# Autodesk Inventor assembly: arm_put_together
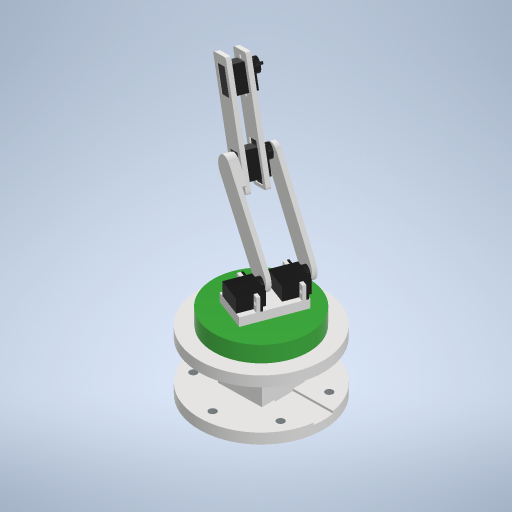
[picture p0: Inventor's stored thumbnail of the model, 512x512]
Saved by Autodesk Inventor 2023 (Build 270158000, 158)
## iProperties
Created: 2023-02-26
Part Number: arm_put_together
Document SubType Name: Assembly
Designer: kamil
Author: kamil
## Documents named in this file (12)
- C:\Users\kamil\Desktop\robotic arm\Inventor_parts\arm_put_together.iam
- C:\Users\kamil\Desktop\robotic arm\Inventor_parts\Base_bottom.ipt
- C:\Users\kamil\Desktop\robotic arm\Inventor_parts\Stepper_model.ipt
- C:\Users\kamil\Desktop\robotic arm\Inventor_parts\Base_top.ipt
- C:\Users\kamil\Desktop\robotic arm\Inventor_parts\Bearing_ball.ipt
- C:\Users\kamil\Desktop\robotic arm\Inventor_parts\Base_arm_mount.ipt
- C:\Users\kamil\Desktop\robotic arm\Inventor_parts\Base_to_servo_mount.ipt
- C:\Users\kamil\Desktop\robotic arm\Inventor_parts\servo_model.ipt
- C:\Users\kamil\Desktop\robotic arm\Inventor_parts\arm_big_part_v1.ipt
- C:\Users\kamil\Desktop\robotic arm\Inventor_parts\arm_big_part_v2.ipt
- C:\Users\kamil\Desktop\robotic arm\Inventor_parts\arm_medium_part_v1.ipt
- C:\Users\kamil\Desktop\robotic arm\Inventor_parts\arm_medium_part_v2.ipt
## Components (37 placed, 11 different names)
1. Base_bottom:1 — Zestawiające:2, Zestawiające:16, Zestawiające:17, Zestawiające:18
2. Stepper_model:1 — Zestawiające:2, Zestawiające:3, Zestawiające:4, Zestawiające:5, Zestawiające:17, Zestawiające:18
3. Base_top:1 — Zestawiające:3, Zestawiające:4, Styczny:1
4. Base_arm_mount:1 — Styczny:2, Zestawiające:5, Zestawiające:6, Zestawiające:7, Zestawiające:8
5. Base_to_servo_mount:1 — Zestawiające:6, Zestawiające:7, Zestawiające:8, Zestawiające:9, Zestawiające:10, Zestawiające:11, Zestawiające:12, Zestawiające:13, Zestawiające:14, Zestawiające:15
6. servo_model:1 — Zestawiające:9, Zestawiające:10, Zestawiające:11, Zestawiające:12, Zestawiające:19, Zestawiające:20
7. servo_model:2 — Zestawiające:13, Zestawiające:14, Zestawiające:15, Zestawiające:21, Zestawiające:22
8. arm_big_part_v1:1 — Zestawiające:19, Zestawiające:20, Zestawiające:23
9. arm_big_part_v2:1 — Zestawiające:21, Zestawiające:22, Zestawiające:29, Zestawiające:30
10. servo_model:3 — Zestawiające:23, Zestawiające:24, Zestawiające:25, Zestawiające:26, Zestawiające:27, Zestawiające:28, Zestawiające:30
11. arm_medium_part_v1:1 — Zestawiające:24, Zestawiające:25, Zestawiające:26, Zestawiające:31, Zestawiające:32, Zestawiające:33
12. arm_medium_part_v2:1 — Zestawiające:27, Zestawiające:28, Zestawiające:29
13. servo_model:4 — Zestawiające:31, Zestawiające:32, Zestawiające:33
14. Bearing_ball:1 — Styczny:1, Styczny:2
15. Bearing_ball:2
16. Bearing_ball:3
17. Bearing_ball:4
18. Bearing_ball:5
19. Bearing_ball:6
20. Bearing_ball:7
21. Bearing_ball:8
22. Bearing_ball:9
23. Bearing_ball:10
24. Bearing_ball:11
25. Bearing_ball:12
26. Bearing_ball:13
27. Bearing_ball:14
28. Bearing_ball:15
29. Bearing_ball:16
30. Bearing_ball:17
31. Bearing_ball:18
32. Bearing_ball:19
33. Bearing_ball:20
34. Bearing_ball:21
35. Bearing_ball:22
36. Bearing_ball:23
37. Bearing_ball:24
## Component patterns: (24 elements, first: Bearing_ball:1)
## Relationships (34: Mate 32, Tangent 2)
- Zestawiające:2 [Mate]: Base_bottom:1 ↔ Stepper_model:1
- Zestawiające:3 [Mate]: Stepper_model:1 ↔ Base_top:1
- Zestawiające:4 [Mate]: Stepper_model:1 ↔ Base_top:1
- Styczny:1 [Tangent]: Base_top:1 ↔ Bearing_ball:1
- Styczny:2 [Tangent]: Base_arm_mount:1 ↔ Bearing_ball:1
- Zestawiające:5 [Mate]: Stepper_model:1 ↔ Base_arm_mount:1
- Zestawiające:6 [Mate]: Base_arm_mount:1 ↔ Base_to_servo_mount:1
- Zestawiające:7 [Mate]: Base_arm_mount:1 ↔ Base_to_servo_mount:1
- Zestawiające:8 [Mate]: Base_arm_mount:1 ↔ Base_to_servo_mount:1
- Zestawiające:9 [Mate]: Base_to_servo_mount:1 ↔ servo_model:1
- Zestawiające:10 [Mate]: Base_to_servo_mount:1 ↔ servo_model:1
- Zestawiające:11 [Mate]: Base_to_servo_mount:1 ↔ servo_model:1
- Zestawiające:12 [Mate]: Base_to_servo_mount:1 ↔ servo_model:1
- Zestawiające:13 [Mate]: Base_to_servo_mount:1 ↔ servo_model:2
- Zestawiające:14 [Mate]: Base_to_servo_mount:1 ↔ servo_model:2
- Zestawiające:15 [Mate]: Base_to_servo_mount:1 ↔ servo_model:2
- Zestawiające:16 [Mate]: Base_bottom:1
- Zestawiające:17 [Mate]: Base_bottom:1 ↔ Stepper_model:1
- Zestawiające:18 [Mate]: Base_bottom:1 ↔ Stepper_model:1
- Zestawiające:19 [Mate]: servo_model:1 ↔ arm_big_part_v1:1
- Zestawiające:20 [Mate]: servo_model:1 ↔ arm_big_part_v1:1
- Zestawiające:21 [Mate]: servo_model:2 ↔ arm_big_part_v2:1
- Zestawiające:22 [Mate]: servo_model:2 ↔ arm_big_part_v2:1
- Zestawiające:23 [Mate]: arm_big_part_v1:1 ↔ servo_model:3
- Zestawiające:24 [Mate]: servo_model:3 ↔ arm_medium_part_v1:1
- Zestawiające:25 [Mate]: servo_model:3 ↔ arm_medium_part_v1:1
- Zestawiające:26 [Mate]: servo_model:3 ↔ arm_medium_part_v1:1
- Zestawiające:27 [Mate]: servo_model:3 ↔ arm_medium_part_v2:1
- Zestawiające:28 [Mate]: servo_model:3 ↔ arm_medium_part_v2:1
- Zestawiające:29 [Mate]: arm_big_part_v2:1 ↔ arm_medium_part_v2:1
- Zestawiające:30 [Mate]: arm_big_part_v2:1 ↔ servo_model:3
- Zestawiające:31 [Mate]: arm_medium_part_v1:1 ↔ servo_model:4
- Zestawiające:32 [Mate]: arm_medium_part_v1:1 ↔ servo_model:4
- Zestawiające:33 [Mate]: arm_medium_part_v1:1 ↔ servo_model:4
